# Autodesk Inventor assembly: A4.1
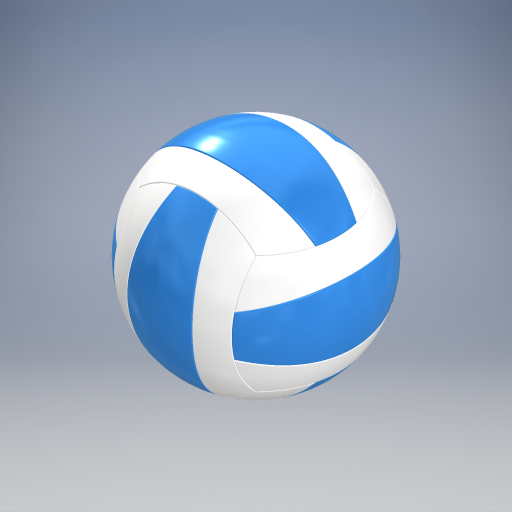
[picture p0: Inventor's stored thumbnail of the model, 512x512]
Saved by Autodesk Inventor 2024 (Build 280153000, 153)
## iProperties
Created: 2024-03-30
Part Number: A4.1
Document SubType Name: Assembly
Designer: Alex
Author: Alex
## Documents named in this file (2)
- C:\Shared\alex-bartella-schoolwork\4z03\Assignment4\A4.1.iam
- C:\Shared\alex-bartella-schoolwork\4z03\Assignment4\subassembly.iam
## Components (6 placed, 1 different names)
1. subassembly:1 [sub-assembly] — Flush:1, Flush:2, Flush:3
2. subassembly:2 [sub-assembly] — Flush:4, Flush:5, Flush:6
3. subassembly:3 [sub-assembly] — Mate:1, Flush:7, Mate:2
4. subassembly:4 [sub-assembly] — Flush:8, Flush:9, Flush:10
5. subassembly:5 [sub-assembly] — Mate:3, Flush:11, Mate:4
6. subassembly:6 [sub-assembly] — Mate:5, Mate:6, Flush:12
## Relationships (18: Flush 12, Mate 6)
- Flush:1: subassembly:1
- Flush:2: subassembly:1
- Flush:3: subassembly:1
- Flush:4: subassembly:2
- Flush:5: subassembly:2
- Flush:6: subassembly:2
- Mate:1: subassembly:3
- Flush:7: subassembly:3
- Mate:2: subassembly:3
- Flush:8: subassembly:4
- Flush:9: subassembly:4
- Flush:10: subassembly:4
- Mate:3: subassembly:5
- Flush:11: subassembly:5
- Mate:4: subassembly:5
- Mate:5: subassembly:6
- Mate:6: subassembly:6
- Flush:12: subassembly:6
